# Autodesk Inventor assembly: Assembly_Total
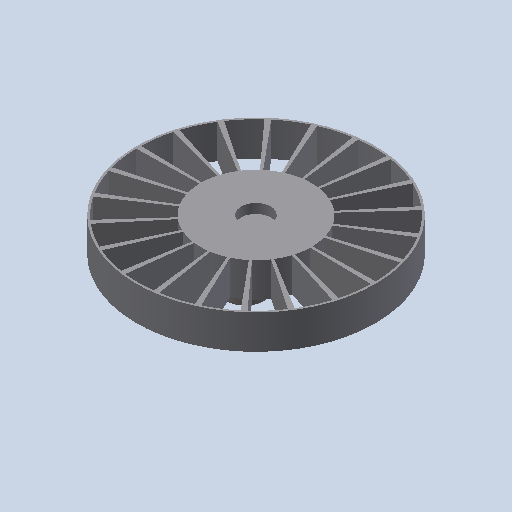
[picture p0: Inventor's stored thumbnail of the model, 512x512]
Saved by Autodesk Inventor 2022 (Build 260153000, 153)
## iProperties
Created: 2023-03-06
Part Number: Assembly_Total
Document SubType Name: Assembly
Designer: zarek
Author: zarek
## Documents named in this file (6)
- C:\Users\zarek\OneDrive\Desktop\Random New Stuff\SPB\Rotational_Piece.iam
- C:\Users\zarek\OneDrive\Desktop\Random New Stuff\SPB\GrabCad Parts\Stepper 28BYJ48.ipt
- C:\Users\zarek\OneDrive\Desktop\Random New Stuff\SPB\Capsule_Design_Revamp.ipt
- C:\Users\zarek\OneDrive\Desktop\Random New Stuff\SPB\Motor_Key_Bearing_2.ipt
- C:\Users\zarek\OneDrive\Desktop\Random New Stuff\SPB\Ball_Bearing_Mock_8_22_7mm.ipt
- C:\Users\zarek\OneDrive\Desktop\Random New Stuff\SPB\Ball_Bearing_Holder.ipt
## Components (5 placed, 5 different names)
1. Stepper 28BYJ48:1 — Rigid:1, Rotational:1
2. Capsule_Design_Revamp:1 — Rigid:2
3. Motor_Key_Bearing_2:1 — Rigid:1, Rigid:2
4. Ball_Bearing_Mock_8_22_7mm:1 — Mate:1
5. Ball_Bearing_Holder:1 — Mate:1, Rotational:1
## Relationships (4: WeldJoint 2, Mate 1, RevoluteJoint 1)
- Rigid:1 [WeldJoint]: Stepper 28BYJ48:1 ↔ Motor_Key_Bearing_2:1
- Rigid:2 [WeldJoint]: Capsule_Design_Revamp:1 ↔ Motor_Key_Bearing_2:1
- Mate:1: Ball_Bearing_Mock_8_22_7mm:1 ↔ Ball_Bearing_Holder:1
- Rotational:1 [RevoluteJoint]: Stepper 28BYJ48:1 ↔ Ball_Bearing_Holder:1
